# Autodesk Inventor assembly: 塔頂組合
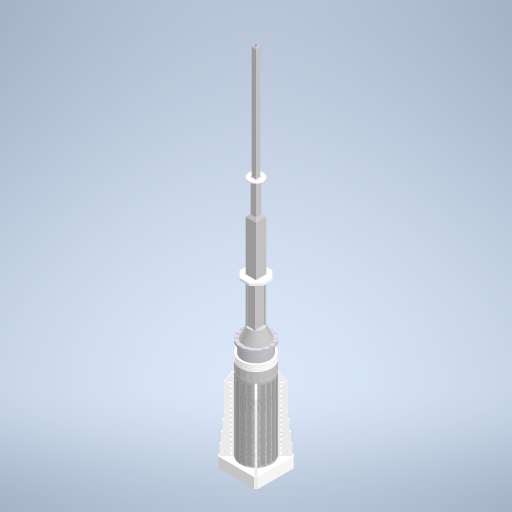
[picture p0: Inventor's stored thumbnail of the model, 512x512]
Saved by Autodesk Inventor 2024.2 (Build 282272000, 272)
## iProperties
Created: 2024-06-05
Part Number: 塔頂組合
Document SubType Name: Assembly
Designer: User
Author: User
## Documents named in this file (8)
- C:\Users\User\OneDrive - 國立中山大學\桌面\創客基礎\final_project\塔頂\塔頂.iam
- C:\Users\User\OneDrive - 國立中山大學\桌面\創客基礎\final_project\塔頂\尖尖.ipt
- C:\Users\User\OneDrive - 國立中山大學\桌面\創客基礎\final_project\塔頂\圓.ipt
- C:\Users\User\OneDrive - 國立中山大學\桌面\創客基礎\final_project\塔頂\盤子上布丁.ipt
- C:\Users\User\OneDrive - 國立中山大學\桌面\創客基礎\final_project\塔頂\援助.ipt
- C:\Users\User\OneDrive - 國立中山大學\桌面\創客基礎\final_project\塔頂\援助上面.ipt
- C:\Users\User\OneDrive - 國立中山大學\桌面\創客基礎\final_project\塔頂\援助旁邊4跟.ipt
- C:\Users\User\OneDrive - 國立中山大學\桌面\創客基礎\final_project\塔頂\樓上跟尖下.ipt
## Components (10 placed, 7 different names)
1. 尖尖:1 — 貼合:1, 貼合:2, 貼合:3
2. 圓:1 — 貼合:4, 貼合:5, 貼合:25
3. 盤子上布丁:1 — 貼合:1, 貼合:2, 貼合:3, 貼合:4, 貼合:5, 貼合:26
4. 援助:1 — 貼合:10, 貼合:11, 貼合:12, 貼合:13, 貼合:14, 貼合:15, 貼合:16, 貼合:17, 齊平:7, 貼合:19, 貼合:20, 齊平:8, 貼合:27
5. 援助上面:1 — 貼合:20, 貼合:25, 貼合:26, 貼合:27
6. 援助旁邊4跟:1 — 貼合:10, 貼合:11, 貼合:24
7. 援助旁邊4跟:2 — 貼合:12, 貼合:13, 貼合:23
8. 援助旁邊4跟:3 — 貼合:14, 貼合:15, 貼合:22
9. 援助旁邊4跟:4 — 貼合:16, 貼合:17, 貼合:21
10. 樓上跟尖下:1 — 齊平:7, 貼合:19, 齊平:8, 貼合:21, 貼合:22, 貼合:23, 貼合:24
## Relationships (24: Mate 22, Flush 2)
- 貼合:1 [Mate]: 尖尖:1 ↔ 盤子上布丁:1
- 貼合:2 [Mate]: 尖尖:1 ↔ 盤子上布丁:1
- 貼合:3 [Mate]: 尖尖:1 ↔ 盤子上布丁:1
- 貼合:4 [Mate]: 圓:1 ↔ 盤子上布丁:1
- 貼合:5 [Mate]: 圓:1 ↔ 盤子上布丁:1
- 貼合:10 [Mate]: 援助:1 ↔ 援助旁邊4跟:1
- 貼合:11 [Mate]: 援助:1 ↔ 援助旁邊4跟:1
- 貼合:12 [Mate]: 援助:1 ↔ 援助旁邊4跟:2
- 貼合:13 [Mate]: 援助:1 ↔ 援助旁邊4跟:2
- 貼合:14 [Mate]: 援助:1 ↔ 援助旁邊4跟:3
- 貼合:15 [Mate]: 援助:1 ↔ 援助旁邊4跟:3
- 貼合:16 [Mate]: 援助:1 ↔ 援助旁邊4跟:4
- 貼合:17 [Mate]: 援助:1 ↔ 援助旁邊4跟:4
- 齊平:7 [Flush]: 援助:1 ↔ 樓上跟尖下:1
- 貼合:19 [Mate]: 援助:1 ↔ 樓上跟尖下:1
- 貼合:20 [Mate]: 援助:1 ↔ 援助上面:1
- 齊平:8 [Flush]: 援助:1 ↔ 樓上跟尖下:1
- 貼合:21 [Mate]: 援助旁邊4跟:4 ↔ 樓上跟尖下:1
- 貼合:22 [Mate]: 援助旁邊4跟:3 ↔ 樓上跟尖下:1
- 貼合:23 [Mate]: 援助旁邊4跟:2 ↔ 樓上跟尖下:1
- 貼合:24 [Mate]: 援助旁邊4跟:1 ↔ 樓上跟尖下:1
- 貼合:25 [Mate]: 圓:1 ↔ 援助上面:1
- 貼合:26 [Mate]: 盤子上布丁:1 ↔ 援助上面:1
- 貼合:27 [Mate]: 援助:1 ↔ 援助上面:1
